# Autodesk Inventor assembly: 横回転ユニット
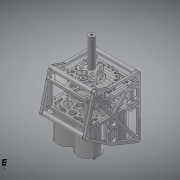
[picture p0: Inventor's stored thumbnail of the model, 180x180]
Saved by Autodesk Inventor 2020 (Build 240168000, 168)
## iProperties
Created: 2019-09-03
Part Number: 横回転ユニット
Material: 一般
Document SubType Name: Assembly
Designer: tanjihayato
Mass: 423.66 g
Surface Area: 689.854 cm^2
Volume: 146.691 cm^3
Density: 2.88812 g/cm^3
Author: tanjihayato
## Documents named in this file (15)
- \\Mac\Home\Documents\Inventor\2019お遊び機体\横回転ユニット.iam
- \\Mac\Home\Documents\Inventor\2019お遊び機体\横回転スライダー.ipt
- \\Mac\Home\Documents\Inventor\2019お遊び機体\横回転最終段.ipt
- \\Mac\Home\Documents\Inventor\2019お遊び機体\横回転最終段カム.ipt
- \\Mac\Home\Documents\Inventor\2019お遊び機体\スペーサ　m3-l6.ipt
- \\Mac\Home\Documents\Inventor\2019お遊び機体\横回転棒取り付けパーツ.ipt
- \\Mac\Home\Documents\Inventor\2019お遊び機体\スペーサ　m4-l45.ipt
- \\Mac\Home\Documents\Inventor\2019お遊び機体\横回転フレーム.ipt
- \\Mac\Home\Documents\Inventor\2019お遊び機体\横回転フレーム２.ipt
- \\Mac\Home\Documents\Inventor\2019お遊び機体\横回転フレーム３.ipt
- \\Mac\Home\Documents\Inventor\2019お遊び機体\モーター(形だけ).ipt
- \\Mac\Home\Documents\Inventor\2019お遊び機体\スペーサ　m3-l20.ipt
- \\Mac\Home\Documents\Inventor\2019お遊び機体\スペーサ　m3-l30.ipt
- \\Mac\Home\Documents\Inventor\2019お遊び機体\横回転フレーム横.ipt
- \\Mac\Home\Documents\Inventor\2019お遊び機体\スペーサ　m3-l55.ipt
## Components (26 placed, 14 different names)
1. 横回転スライダー:1 — 挿入:2, 挿入:5, メイト:1
2. 横回転最終段:1 — 挿入:1, 挿入:2, 挿入:3
3. 横回転最終段カム:1 — 挿入:1, 挿入:4, 挿入:7, メイト:2
4. スペーサ　m3-l6:1 — 挿入:4
5. スペーサ　m3-l6:2 — 挿入:3
6. 横回転棒取り付けパーツ:1 — 挿入:5, メイト:1, 挿入:6
7. スペーサ　m4-l45:1 — 挿入:6
8. 横回転フレーム:1 — 挿入:7, メイト:2, 挿入:8, 挿入:9, 挿入:15, 挿入:16
9. 横回転フレーム２:1 — 挿入:10, メイト:3, 挿入:18, 挿入:19
10. スペーサ　m3-l6:3 — 挿入:8, メイト:3
11. スペーサ　m3-l6:4 — 挿入:9, 挿入:10
12. 横回転フレーム３:1 — 挿入:11, 挿入:12, 挿入:13, 挿入:14, 挿入:17, メイト:4, フラッシュ:1, メイト:5, メイト:6, フラッシュ:2, メイト:7, メイト:8
13. モーター(形だけ):1 — 挿入:11
14. モーター(形だけ):2 — 挿入:12
15. モーター(形だけ):3 — 挿入:13
16. モーター(形だけ):4 — 挿入:14
17. スペーサ　m3-l20:1 — 挿入:15, 挿入:17
18. スペーサ　m3-l20:2 — 挿入:16, メイト:4
19. スペーサ　m3-l30:1 — 挿入:18
20. スペーサ　m3-l30:2 — 挿入:19
21. 横回転フレーム横:1 — フラッシュ:1, メイト:5, メイト:6
22. 横回転フレーム横:2 — フラッシュ:2, メイト:7, メイト:8, 挿入:20, 挿入:21, 挿入:22, 挿入:23
23. スペーサ　m3-l55:1 — 挿入:20
24. スペーサ　m3-l55:2 — 挿入:22
25. スペーサ　m3-l55:3 — 挿入:21
26. スペーサ　m3-l55:4 — 挿入:23
## Relationships (33: Insert 23, Mate 8, Flush 2)
- 挿入:1 [Insert]: 横回転最終段:1 ↔ 横回転最終段カム:1
- 挿入:2 [Insert]: 横回転スライダー:1 ↔ 横回転最終段:1
- 挿入:3 [Insert]: 横回転最終段:1 ↔ スペーサ　m3-l6:2
- 挿入:4 [Insert]: 横回転最終段カム:1 ↔ スペーサ　m3-l6:1
- 挿入:5 [Insert]: 横回転スライダー:1 ↔ 横回転棒取り付けパーツ:1
- メイト:1 [Mate]: 横回転スライダー:1 ↔ 横回転棒取り付けパーツ:1
- 挿入:6 [Insert]: 横回転棒取り付けパーツ:1 ↔ スペーサ　m4-l45:1
- 挿入:7 [Insert]: 横回転最終段カム:1 ↔ 横回転フレーム:1
- メイト:2 [Mate]: 横回転最終段カム:1 ↔ 横回転フレーム:1
- 挿入:8 [Insert]: 横回転フレーム:1 ↔ スペーサ　m3-l6:3
- 挿入:9 [Insert]: 横回転フレーム:1 ↔ スペーサ　m3-l6:4
- 挿入:10 [Insert]: 横回転フレーム２:1 ↔ スペーサ　m3-l6:4
- メイト:3 [Mate]: 横回転フレーム２:1 ↔ スペーサ　m3-l6:3
- 挿入:11 [Insert]: 横回転フレーム３:1 ↔ モーター(形だけ):1
- 挿入:12 [Insert]: 横回転フレーム３:1 ↔ モーター(形だけ):2
- 挿入:13 [Insert]: 横回転フレーム３:1 ↔ モーター(形だけ):3
- 挿入:14 [Insert]: 横回転フレーム３:1 ↔ モーター(形だけ):4
- 挿入:15 [Insert]: 横回転フレーム:1 ↔ スペーサ　m3-l20:1
- 挿入:16 [Insert]: 横回転フレーム:1 ↔ スペーサ　m3-l20:2
- 挿入:17 [Insert]: 横回転フレーム３:1 ↔ スペーサ　m3-l20:1
- メイト:4 [Mate]: 横回転フレーム３:1 ↔ スペーサ　m3-l20:2
- 挿入:18 [Insert]: 横回転フレーム２:1 ↔ スペーサ　m3-l30:1
- 挿入:19 [Insert]: 横回転フレーム２:1 ↔ スペーサ　m3-l30:2
- フラッシュ:1 [Flush]: 横回転フレーム３:1 ↔ 横回転フレーム横:1
- メイト:5 [Mate]: 横回転フレーム３:1 ↔ 横回転フレーム横:1
- メイト:6 [Mate]: 横回転フレーム３:1 ↔ 横回転フレーム横:1
- フラッシュ:2 [Flush]: 横回転フレーム３:1 ↔ 横回転フレーム横:2
- メイト:7 [Mate]: 横回転フレーム３:1 ↔ 横回転フレーム横:2
- メイト:8 [Mate]: 横回転フレーム３:1 ↔ 横回転フレーム横:2
- 挿入:20 [Insert]: 横回転フレーム横:2 ↔ スペーサ　m3-l55:1
- 挿入:21 [Insert]: 横回転フレーム横:2 ↔ スペーサ　m3-l55:3
- 挿入:22 [Insert]: 横回転フレーム横:2 ↔ スペーサ　m3-l55:2
- 挿入:23 [Insert]: 横回転フレーム横:2 ↔ スペーサ　m3-l55:4
